# Autodesk Inventor assembly: 50mm_EDF
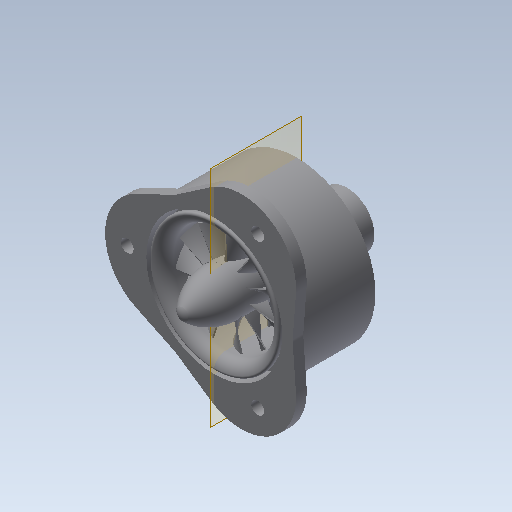
[picture p0: Inventor's stored thumbnail of the model, 512x512]
Saved by Autodesk Inventor 2020 (Build 240168000, 168)
## iProperties
Created: 2017-11-27
Part Number: 50mm_EDF
Document SubType Name: Assembly
Designer: USER
Author: USER
## Documents named in this file (6)
- E:\MENG Project\Open-AMR-Hardware\Hardware\MCAD\EDF\50mm_EDF.iam
- E:\MENG Project\Open-AMR-Hardware\Hardware\MCAD\EDF\motor.ipt
- E:\MENG Project\Open-AMR-Hardware\Hardware\MCAD\EDF\風扇本體.ipt
- E:\MENG Project\Open-AMR-Hardware\Hardware\MCAD\EDF\風扇頭.ipt
- E:\MENG Project\Open-AMR-Hardware\Hardware\MCAD\EDF\扇葉.ipt
- E:\MENG Project\Open-AMR-Hardware\Hardware\MCAD\EDF\EDF Mount.ipt
## Components (5 placed, 5 different names)
1. motor:1 — 貼合:1, 貼合:2, 旋轉:1, Mate:8
2. 風扇本體:1 — 貼合:1, 貼合:2, 貼合:3, 貼合:4, 旋轉:2, Mate:9
3. 風扇頭:1 — 貼合:3, 貼合:4, 貼合:5, 貼合:6, 貼合:7, 旋轉:2
4. 扇葉:1 — 貼合:5, 貼合:6, 旋轉:1
5. EDF Mount:1 — Mate:8, Mate:9
## Relationships (11: Mate 9, RelateRotation 2)
- 貼合:1 [Mate]: motor:1 ↔ 風扇本體:1
- 貼合:2 [Mate]: motor:1 ↔ 風扇本體:1
- 貼合:3 [Mate]: 風扇本體:1 ↔ 風扇頭:1
- 貼合:4 [Mate] (-3.7 mm): 風扇本體:1 ↔ 風扇頭:1
- 貼合:5 [Mate]: 風扇頭:1 ↔ 扇葉:1
- 貼合:6 [Mate]: 風扇頭:1 ↔ 扇葉:1
- 貼合:7 [Mate]: 風扇頭:1
- 旋轉:1 [RelateRotation] (0.844 ul): motor:1 ↔ 扇葉:1
- 旋轉:2 [RelateRotation] (1 ul): 風扇本體:1 ↔ 風扇頭:1
- Mate:8: motor:1 ↔ EDF Mount:1
- Mate:9: 風扇本體:1 ↔ EDF Mount:1
